# Autodesk Inventor assembly: z-keeper-asm
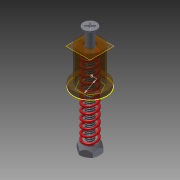
[picture p0: Inventor's stored thumbnail of the model, 180x180]
Saved by Autodesk Inventor 2014 (Build 180170000, 170)
## iProperties
Created: 2014-01-09
Part Number: z-keeper-asm
Document SubType Name: Assembly
Designer: caleb
Author: caleb
## Documents named in this file (5)
- C:\cygwin\home\caleb\caleb-typea-settings\designs\z-lead-screw-keeper\z-keeper-asm.iam
- C:\cygwin\home\caleb\caleb-typea-settings\designs\z-lead-screw-keeper\z-keeper.ipt
- C:\Documents and Settings\caleb\My Documents\Inventor\Content Center Files\R2014\en-US\IFI 100 107(2)\IFI 100_107 - No. 6 - 32 Top Insert Type.ipt
- C:\Documents and Settings\caleb\My Documents\Inventor\Content Center Files\R2014\en-US\ANSI B18.6.3(00)\ANSI B18.6.3 - 6-32 UNC - 2(32).ipt
- C:\cygwin\home\caleb\caleb-typea-settings\designs\z-lead-screw-keeper\spring.ipt
## Components (4 placed, 4 different names)
1. z-keeper:1 — Mate:1, Mate:3, Mate:4, Mate:5
2. Prevailing Torque Type Hex Nut - Inch (IFI) No. 6 - 32 Top Insert Type:1 — Mate:2
3. Cross Recessed 100° Flat Countersunk Head Machine Screw - Type I - Inch 6-32 UNC x 2:1 — Mate:1, Mate:2, Mate:3, Mate:6
4. spring:1 — Mate:6
## Relationships (6: Mate 6)
- Mate:1: z-keeper:1 ↔ Cross Recessed 100° Flat Countersunk Head Machine Screw - Type I - Inch 6-32 UNC x 2:1
- Mate:2: Prevailing Torque Type Hex Nut - Inch (IFI) No. 6 - 32 Top Insert Type:1 ↔ Cross Recessed 100° Flat Countersunk Head Machine Screw - Type I - Inch 6-32 UNC x 2:1
- Mate:3: z-keeper:1 ↔ Cross Recessed 100° Flat Countersunk Head Machine Screw - Type I - Inch 6-32 UNC x 2:1
- Mate:4: z-keeper:1
- Mate:5: z-keeper:1
- Mate:6: Cross Recessed 100° Flat Countersunk Head Machine Screw - Type I - Inch 6-32 UNC x 2:1 ↔ spring:1
